# Autodesk Inventor assembly: rocket_asm
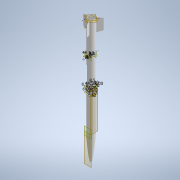
[picture p0: Inventor's stored thumbnail of the model, 180x180]
Saved by Autodesk Inventor 2020 (Build 240168000, 168)
## iProperties
Created: 2022-06-15
Part Number: rocket_asm
Document SubType Name: Assembly
Designer: sp
Author: sp
## Documents named in this file (13)
- C:\Users\sp\Documents\Rocket\rocket\CAD\rocket_asm.iam
- C:\Users\sp\Documents\Rocket\rocket\CAD\Engine.ipt
- C:\Users\sp\Documents\Rocket\rocket\CAD\Segment_elektro.ipt
- C:\Users\sp\Documents\Rocket\rocket\CAD\Segment_Engine.ipt
- C:\Users\sp\Documents\Rocket\rocket\CAD\Segment_recovery.ipt
- C:\Users\sp\Documents\Rocket\rocket\CAD\Spitze.ipt
- C:\Users\sp\Documents\Rocket\rocket\CAD\Leitwerk.ipt
- C:\Users\sp\Documents\Rocket\rocket\CAD\Back_holder.ipt
- C:\Users\sp\Documents\Rocket\rocket\CAD\Ronde_Engine.ipt
- C:\Users\sp\Documents\Rocket\rocket\CAD\recovery_asm.iam
- C:\Users\sp\Documents\Rocket\rocket\CAD\servo_asm.iam
- C:\Users\sp\Documents\Rocket\rocket\CAD\Deckel_Parachute_6.ipt
- C:\Users\sp\Documents\Rocket\rocket\CAD\Cam_konstruction.ipt
## Components (14 placed, 12 different names)
1. Engine:1 — Passend:1, Einfügen:1, Einfügen:2, Passend:2, Einfügen:3
2. Segment_elektro:1 — Einfügen:8, Einfügen:9
3. Segment_Engine:1 — Einfügen:2, Passend:3, Passend:4, Passend:5, Passend:6, Passend:7, Passend:8, Einfügen:4
4. Segment_recovery:1 — Einfügen:5, Fluchtend:1, Einfügen:6
5. Spitze:1 — Einfügen:10
6. Leitwerk:1 — Passend:7, Passend:8
7. Leitwerk:2 — Passend:3, Passend:4
8. Leitwerk:3 — Passend:5, Passend:6
9. Back_holder:1 — Passend:2, Einfügen:3
10. Ronde_Engine:1 — Passend:1, Einfügen:1
11. recovery_asm:1 [sub-assembly] — Einfügen:4, Einfügen:5, Fluchtend:1, Einfügen:7
12. servo_asm:1 [sub-assembly] — Einfügen:6, Einfügen:8
13. Deckel_Parachute_6:1 — Einfügen:7
14. Cam_konstruction:1 — Einfügen:9, Einfügen:10
## Relationships (19: Insert 10, Mate 8, Flush 1)
- Passend:1 [Mate]: Engine:1 ↔ Ronde_Engine:1
- Einfügen:1 [Insert]: Engine:1 ↔ Ronde_Engine:1
- Einfügen:2 [Insert]: Engine:1 ↔ Segment_Engine:1
- Passend:2 [Mate]: Engine:1 ↔ Back_holder:1
- Einfügen:3 [Insert]: Engine:1 ↔ Back_holder:1
- Passend:3 [Mate]: Segment_Engine:1 ↔ Leitwerk:2
- Passend:4 [Mate]: Segment_Engine:1 ↔ Leitwerk:2
- Passend:5 [Mate]: Segment_Engine:1 ↔ Leitwerk:3
- Passend:6 [Mate]: Segment_Engine:1 ↔ Leitwerk:3
- Passend:7 [Mate]: Segment_Engine:1 ↔ Leitwerk:1
- Passend:8 [Mate]: Segment_Engine:1 ↔ Leitwerk:1
- Einfügen:4 [Insert]: Segment_Engine:1 ↔ recovery_asm:1
- Einfügen:5 [Insert]: Segment_recovery:1 ↔ recovery_asm:1
- Fluchtend:1 [Flush]: Segment_recovery:1 ↔ recovery_asm:1
- Einfügen:6 [Insert]: Segment_recovery:1 ↔ servo_asm:1
- Einfügen:7 [Insert] (-73 mm): recovery_asm:1 ↔ Deckel_Parachute_6:1
- Einfügen:8 [Insert]: Segment_elektro:1 ↔ servo_asm:1
- Einfügen:9 [Insert]: Segment_elektro:1 ↔ Cam_konstruction:1
- Einfügen:10 [Insert]: Spitze:1 ↔ Cam_konstruction:1
